# Autodesk Inventor assembly: Assembly
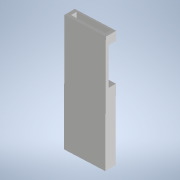
[picture p0: Inventor's stored thumbnail of the model, 180x180]
Saved by Autodesk Inventor 2020 (Build 240168000, 168)
## iProperties
Created: 2020-06-06
Part Number: Assembly
Document SubType Name: Assembly
Designer: user
Author: user
## Documents named in this file (4)
- C:\Users\user\Desktop\GateClip\Assembly.iam
- C:\Users\user\Desktop\GateClip\Clip.ipt
- C:\Users\user\Desktop\GateClip\End.ipt
- C:\Users\user\Desktop\GateClip\Middle.ipt
## Components (4 placed, 3 different names)
1. BodyEnd:1 — Mate:1, Flush:1, Flush:2, Flush:3, Flush:13, Flush:16, Flush:17
2. Clip:1 — Mate:1, Flush:1, Flush:2, Flush:3, Mate:2, Flush:5, Flush:6, Flush:7, Flush:8, Flush:13, Flush:15, Flush:16, Flush:17
3. Middle:1 — Mate:2, Flush:5, Flush:6, Flush:7, Flush:8, Mate:3, Flush:9, Flush:10, Flush:11, Flush:12, Flush:15
4. Clip:2 — Mate:3, Flush:9, Flush:10, Flush:11, Flush:12
## Relationships (18: Flush 15, Mate 3)
- Mate:1: BodyEnd:1 ↔ Clip:1
- Flush:1: BodyEnd:1 ↔ Clip:1
- Flush:2: BodyEnd:1 ↔ Clip:1
- Flush:3: BodyEnd:1 ↔ Clip:1
- Mate:2: Clip:1 ↔ Middle:1
- Flush:5: Clip:1 ↔ Middle:1
- Flush:6: Clip:1 ↔ Middle:1
- Flush:7: Clip:1 ↔ Middle:1
- Flush:8: Clip:1 ↔ Middle:1
- Mate:3: Middle:1 ↔ Clip:2
- Flush:9: Middle:1 ↔ Clip:2
- Flush:10: Middle:1 ↔ Clip:2
- Flush:11: Middle:1 ↔ Clip:2
- Flush:12: Middle:1 ↔ Clip:2
- Flush:13: BodyEnd:1 ↔ Clip:1
- Flush:15: Clip:1 ↔ Middle:1
- Flush:16: BodyEnd:1 ↔ Clip:1
- Flush:17: BodyEnd:1 ↔ Clip:1
